# Autodesk Inventor assembly: VWheel
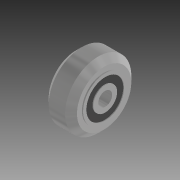
[picture p0: Inventor's stored thumbnail of the model, 180x180]
Saved by Autodesk Inventor 2020 (Build 240168000, 168)
## iProperties
Created: 2020-10-19
Part Number: VWheel
Document SubType Name: Assembly
Designer: DDeGo
Author: DDeGo
## Documents named in this file (3)
- C:\Users\DDeGo\Documents\Drew\Projects\De-Cruster\cad\VWheel.iam
- C:\Users\DDeGo\Documents\Drew\Projects\De-Cruster\cad\Ball Bearing 5 x 16 x 5 v1.ipt
- C:\Users\DDeGo\Documents\Drew\Projects\De-Cruster\cad\Xtreme Solid V Wheel v1.ipt
## Components (3 placed, 2 different names)
1. Ball Bearing 5 x 16 x 5 v1:1 — Mate:2, Mate:3
2. Xtreme Solid V Wheel v1:1 — Mate:1, Mate:2, Mate:3, Mate:4
3. Ball Bearing 5 x 16 x 5 v1:2 — Mate:1, Mate:4
## Relationships (4: Mate 4)
- Mate:1: Xtreme Solid V Wheel v1:1 ↔ Ball Bearing 5 x 16 x 5 v1:2
- Mate:2: Ball Bearing 5 x 16 x 5 v1:1 ↔ Xtreme Solid V Wheel v1:1
- Mate:3: Ball Bearing 5 x 16 x 5 v1:1 ↔ Xtreme Solid V Wheel v1:1
- Mate:4: Xtreme Solid V Wheel v1:1 ↔ Ball Bearing 5 x 16 x 5 v1:2
